# Autodesk Inventor assembly: RealSenseD543Assembly
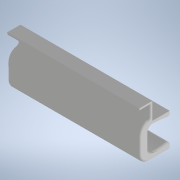
[picture p0: Inventor's stored thumbnail of the model, 180x180]
Saved by Autodesk Inventor 2021 (Build 250183000, 183)
## iProperties
Created: 2021-05-13
Part Number: RealSenseD543Assembly
Document SubType Name: Assembly
Designer: gisen
Author: gisen
## Documents named in this file (3)
- D:\GitProjects\CAD-Data\Devices\RealSenseD435\RealSenseD543Assembly.iam
- D:\GitProjects\CAD-Data\Devices\RealSenseD435\RealSenseD435.iam
- D:\GitProjects\CAD-Data\Devices\RealSenseD435\RealSenseD435Cradle.ipt
## Components (2 placed, 2 different names)
1. RealSenseD435:1 [sub-assembly] — フラッシュ:3, フラッシュ:4, フラッシュ:5
2. RealSenseD435Cradle:1 — フラッシュ:1, フラッシュ:2, フラッシュ:4, フラッシュ:5
## Relationships (5: Flush 5)
- フラッシュ:1 [Flush]: RealSenseD435Cradle:1
- フラッシュ:2 [Flush]: RealSenseD435Cradle:1
- フラッシュ:3 [Flush] (-18 mm): RealSenseD435:1
- フラッシュ:4 [Flush] (-3 mm): RealSenseD435:1 ↔ RealSenseD435Cradle:1
- フラッシュ:5 [Flush] (65 mm): RealSenseD435:1 ↔ RealSenseD435Cradle:1
